# Autodesk Inventor assembly: Ankle_side_pitch
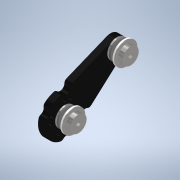
[picture p0: Inventor's stored thumbnail of the model, 180x180]
Saved by Autodesk Inventor 2022.3 (Build 263350000, 350)
## iProperties
Created: 2022-06-04
Part Number: Ankle_side_pitch
Document SubType Name: Assembly
Designer: Masato Kubotera
Author: Masato Kubotera
## Documents named in this file (10)
- C:\Users\Masato\Desktop\SUSTAINA-OP\LowerBody\Ankle\Ankle_side_pitch.iam
- C:\Users\Masato\Desktop\SUSTAINA-OP\LowerBody\Ankle\Ankle_side_pitch_frame.ipt
- C:\Users\Masato\Desktop\SUSTAINA-OP\ReadyMade\InsertNut\S4-05-3W.ipt
- C:\Users\Masato\Desktop\SUSTAINA-OP\ReadyMade\InsertNut\SF419.ipt
- C:\Users\Masato\Desktop\SUSTAINA-OP\ReadyMade\Washer\UUW-0412-10H.ipt
- C:\Users\Masato\Desktop\SUSTAINA-OP\ReadyMade\Bush\80F-0603.ipt
- C:\Users\Masato\Desktop\SUSTAINA-OP\ReadyMade\Washer\TT-0814-10.ipt
- C:\Users\Masato\Desktop\SUSTAINA-OP\ReadyMade\Washer\UUW-0614-03H.ipt
- C:\Users\Masato\Desktop\SUSTAINA-OP\ReadyMade\Screw\DBTS4-4.5-5-DHC-LTC.ipt
- C:\Users\Masato\Desktop\SUSTAINA-OP\ReadyMade\Screw\DBTS4-4.5-5-DHC-LTC_mod.ipt
## Components (13 placed, 9 different names)
1. Ankle_side_pitch_frame:1 — メイト:1, 角度:1, メイト:2, 挿入:1, 挿入:2, 挿入:3, 挿入:4
2. UUW-0614-03H:2 — 挿入:10, 挿入:12
3. UUW-0614-03H:1 — 挿入:9, 挿入:11
4. TT-0814-10:2 — 挿入:12
5. TT-0814-10:1 — 挿入:11
6. 80F-0603:2 — 挿入:6
7. 80F-0603:1 — 挿入:5
8. UUW-0412-10H:2 — 挿入:4, 挿入:6, 挿入:8
9. UUW-0412-10H:1 — 挿入:3, 挿入:5, 挿入:7
10. SF419:1 — 挿入:2
11. S4-05-3W:1 — 挿入:1
12. DBTS4-4.5-5-DHC-LTC:1 — 挿入:8, 挿入:10
13. DBTS4-4.5-5-DHC-LTC_mod:1 — 挿入:7, 挿入:9
## Relationships (15: Insert 12, Mate 2, Angle 1)
- メイト:1 [Mate] (25.25 mm): Ankle_side_pitch_frame:1
- 角度:1 [Angle] (147.9946 deg): Ankle_side_pitch_frame:1
- メイト:2 [Mate]: Ankle_side_pitch_frame:1
- 挿入:1 [Insert]: Ankle_side_pitch_frame:1 ↔ S4-05-3W:1
- 挿入:2 [Insert]: Ankle_side_pitch_frame:1 ↔ SF419:1
- 挿入:3 [Insert]: Ankle_side_pitch_frame:1 ↔ UUW-0412-10H:1
- 挿入:4 [Insert]: Ankle_side_pitch_frame:1 ↔ UUW-0412-10H:2
- 挿入:5 [Insert]: 80F-0603:1 ↔ UUW-0412-10H:1
- 挿入:6 [Insert]: 80F-0603:2 ↔ UUW-0412-10H:2
- 挿入:7 [Insert]: UUW-0412-10H:1 ↔ DBTS4-4.5-5-DHC-LTC_mod:1
- 挿入:8 [Insert]: UUW-0412-10H:2 ↔ DBTS4-4.5-5-DHC-LTC:1
- 挿入:9 [Insert]: UUW-0614-03H:1 ↔ DBTS4-4.5-5-DHC-LTC_mod:1
- 挿入:10 [Insert]: UUW-0614-03H:2 ↔ DBTS4-4.5-5-DHC-LTC:1
- 挿入:11 [Insert]: UUW-0614-03H:1 ↔ TT-0814-10:1
- 挿入:12 [Insert]: UUW-0614-03H:2 ↔ TT-0814-10:2
